# Autodesk Inventor assembly: BG005_trajan20_21
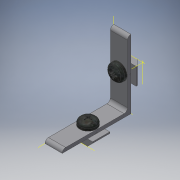
[picture p0: Inventor's stored thumbnail of the model, 180x180]
Saved by Autodesk Inventor 2022.2 (Build 262287000, 287)
## iProperties
Company: HTBLA Kaindorf
RuleStatus: InUse
Created: 2022-06-22
Part Number: BG005_trajan20_21
Project: Zeichenmaschine_v2
Material: Generisch
Description: winkel
Document SubType Name: Assembly
Designer: trajan20
AfterDocNew0: iProperties-Editor_aufrufen
Author: jan
Keywords: 2021
## Documents named in this file (4)
- C:\Users\jan\Documents\DrawMachine\DrawMachineConstruction\Projekt\Zeichenmaschine_v2\BG005_trajan20_21_Zeichenmaschine_v2_winkel.iam
- C:\Users\jan\Documents\DrawMachine\DrawMachineConstruction\Projekt\Zeichenmaschine_v2\BTwinkel1_trajan20_21_Zeichenmaschine_v2_profil.ipt
- C:\Users\jan\Documents\DrawMachine\DrawMachineConstruction\Projekt\Zeichenmaschine_v2\BTwnikel2_trajan20_21_Zeichenmaschine_v2_nutenstein.ipt
- C:\Users\jan\Documents\DrawMachine\DrawMachineConstruction\Projekt\Zeichenmaschine_v2\Normteile\de-DE\ISO 7045  Z\ISO 7045 - M5 x 8_ - 4.8 - Z - ISO.ipt
## Components (5 placed, 3 different names)
1. BTwinkel1_trajan20_21_Zeichenmaschine_v2_profil:1 — Passend:1, Passend:2, Passend:3, Passend:4, Passend:5, Passend:6, Passend:7
2. BTwnikel2_trajan20_21_Zeichenmaschine_v2_nutenstein:1 — Passend:1, Passend:2, Passend:8
3. BTwnikel2_trajan20_21_Zeichenmaschine_v2_nutenstein:2 — Passend:3, Passend:4
4. ISO 7045 Z M5 x 8 - 4.8 - Z:1 — Passend:5, Passend:6
5. ISO 7045 Z M5 x 8 - 4.8 - Z:2 — Passend:7, Passend:8
## Relationships (8: Mate 8)
- Passend:1 [Mate]: BTwinkel1_trajan20_21_Zeichenmaschine_v2_profil:1 ↔ BTwnikel2_trajan20_21_Zeichenmaschine_v2_nutenstein:1
- Passend:2 [Mate]: BTwinkel1_trajan20_21_Zeichenmaschine_v2_profil:1 ↔ BTwnikel2_trajan20_21_Zeichenmaschine_v2_nutenstein:1
- Passend:3 [Mate]: BTwinkel1_trajan20_21_Zeichenmaschine_v2_profil:1 ↔ BTwnikel2_trajan20_21_Zeichenmaschine_v2_nutenstein:2
- Passend:4 [Mate]: BTwinkel1_trajan20_21_Zeichenmaschine_v2_profil:1 ↔ BTwnikel2_trajan20_21_Zeichenmaschine_v2_nutenstein:2
- Passend:5 [Mate]: BTwinkel1_trajan20_21_Zeichenmaschine_v2_profil:1 ↔ ISO 7045 Z M5 x 8 - 4.8 - Z:1
- Passend:6 [Mate]: BTwinkel1_trajan20_21_Zeichenmaschine_v2_profil:1 ↔ ISO 7045 Z M5 x 8 - 4.8 - Z:1
- Passend:7 [Mate]: BTwinkel1_trajan20_21_Zeichenmaschine_v2_profil:1 ↔ ISO 7045 Z M5 x 8 - 4.8 - Z:2
- Passend:8 [Mate]: BTwnikel2_trajan20_21_Zeichenmaschine_v2_nutenstein:1 ↔ ISO 7045 Z M5 x 8 - 4.8 - Z:2
